# Autodesk Inventor assembly: VersaPlanetary_v2_Two_Stage_100_1_with_BAG
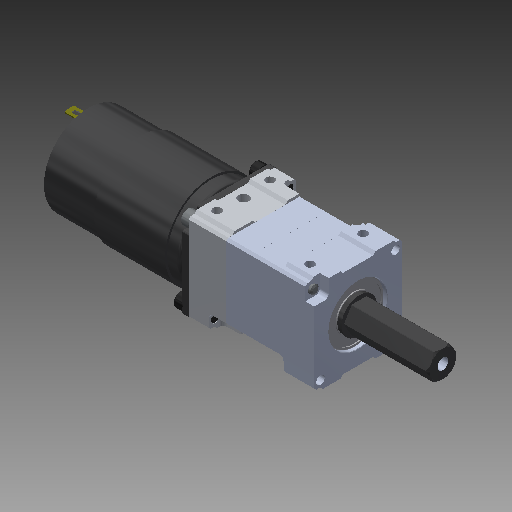
[picture p0: Inventor's stored thumbnail of the model, 512x512]
Saved by Autodesk Inventor 2018 (Build 220112000, 112)
## iProperties
Created: 2016-10-31
Part Number: VersaPlanetary_v2_Two_Stage_100_1_with_BAG
Description: STEP AP214
Document SubType Name: Assembly
Designer: collostr18
Sending System: SolidWorks 2016
Preprocessor: SwSTEP 2.0
Title: 217-4973_2stage_BAG.STEP
Revision Number: ANY
## Documents named in this file (17)
- D:\Lift for Box\STEPS\2 Stage VP with 775pro\VersaPlanetary_v2_Two_Stage_100_1_with_BAG.iam
- D:\Lift for Box\STEPS\2 Stage VP with 775pro\217-2625-026 Rev1.ipt
- D:\Lift for Box\STEPS\2 Stage VP with 775pro\217-2742-001 Rev4.ipt
- D:\Lift for Box\STEPS\2 Stage VP with 775pro\217-2625-017 Rev1_9714K61.ipt
- D:\Lift for Box\STEPS\2 Stage VP with 775pro\217-2625-003 Rev1.ipt
- D:\Lift for Box\STEPS\2 Stage VP with 775pro\217-2625-018 Rev1_98541A410.ipt
- D:\Lift for Box\STEPS\2 Stage VP with 775pro\832-2250-Base-Kit-Screw_SSA0832-0500ZC.ipt
- D:\Lift for Box\STEPS\2 Stage VP with 775pro\217-2625-025 Rev1.ipt
- D:\Lift for Box\STEPS\2 Stage VP with 775pro\217-4649-002 Rev1_SSA0832-0500ZC.ipt
- D:\Lift for Box\STEPS\2 Stage VP with 775pro\217-4649-006 Rev1_SSA0004-008BA.ipt
- D:\Lift for Box\STEPS\2 Stage VP with 775pro\217-2822-003 Rev4.ipt
- D:\Lift for Box\STEPS\2 Stage VP with 775pro\217-2820 Rev1_Public.iam
- D:\Lift for Box\STEPS\2 Stage VP with 775pro\217-2816-001 Rev1.ipt
- D:\Lift for Box\STEPS\2 Stage VP with 775pro\217-4649-001 Rev1.ipt
- D:\Lift for Box\STEPS\2 Stage VP with 775pro\217-4649-007 Rev1_94105A824.ipt
- D:\Lift for Box\STEPS\2 Stage VP with 775pro\217-2625-011 Rev1.ipt
- D:\Lift for Box\STEPS\2 Stage VP with 775pro\775pro_217-4347.ipt
## Components (22 placed, 22 different names)
1. 217-2625-026 Rev1_1
2. 217-2742-001 Rev4_2
3. 217-2742-001 Rev4_3
4. 217-2625-017 Rev1_9714K61_4
5. 217-2625-003 Rev1_5
6. 217-2625-018 Rev1_98541A410_6
7. 832-2250-Base-Kit-Screw_SSA0832-0500ZC_7
8. 832-2250-Base-Kit-Screw_SSA0832-0500ZC_8
9. 217-2625-025 Rev1_9
10. 217-4649-002 Rev1_SSA0832-0500ZC_10
11. 217-4649-002 Rev1_SSA0832-0500ZC_11
12. 217-4649-006 Rev1_SSA0004-008BA_12
13. 217-4649-006 Rev1_SSA0004-008BA_13
14. 217-2822-003 Rev4_14 — Mate:1, Mate:2
15. 217-2820 Rev1_Public_16 [sub-assembly]
16. 217-2816-001 Rev1_17
17. 217-2820 Rev1_Public_18 [sub-assembly]
18. 217-2816-001 Rev1_19
19. 217-4649-001 Rev1_20
20. 217-4649-007 Rev1_94105A824_21
21. 217-2625-011 Rev1_22
22. 775pro_217-4347:1 — Mate:1, Mate:2
## Relationships (2: Mate 2)
- Mate:1: 217-2822-003 Rev4_14 ↔ 775pro_217-4347:1
- Mate:2: 217-2822-003 Rev4_14 ↔ 775pro_217-4347:1
